# Autodesk Inventor assembly: Gyro
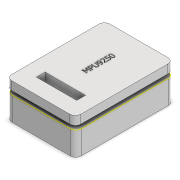
[picture p0: Inventor's stored thumbnail of the model, 180x180]
Saved by Autodesk Inventor 2020 (Build 240168000, 168)
## iProperties
Created: 2019-08-08
Part Number: Gyro
Document SubType Name: Assembly
Designer: chitl
Author: chitl
## Documents named in this file (5)
- C:\Users\chitl\Desktop\OneWheel\Wheel Assembled\Electronics\Gyro.iam
- C:\Users\chitl\Desktop\OneWheel\Wheel Assembled\Electronics\Gyro.ipt
- C:\Users\chitl\Desktop\OneWheel\Wheel Assembled\Electronics\JST Socket 6 Pin.ipt
- C:\Users\chitl\Desktop\OneWheel\Wheel Assembled\Electronics\Gyro_box_bottom.ipt
- C:\Users\chitl\Desktop\OneWheel\Wheel Assembled\Electronics\Gyro_box_Top.ipt
## Components (4 placed, 4 different names)
1. Gyro:1 — Mate:1
2. JST Socket 6 Pin:1
3. Gyro_box_bottom:1 — Mate:1
4. Gyro_box_Top:1
## Relationships (1: Mate 1)
- Mate:1: Gyro:1 ↔ Gyro_box_bottom:1
